# Autodesk Inventor assembly: assembly
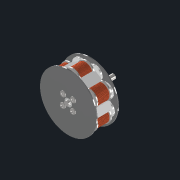
[picture p0: Inventor's stored thumbnail of the model, 180x180]
Saved by Autodesk Inventor 2022.2 (Build 262287010, 287A)
## iProperties
Created: 2023-07-19
Part Number: assembly
Document SubType Name: Assembly
Designer: StijnC
Author: StijnC
## Documents named in this file (10)
- C:\Users\techn\Desktop\AFM\V2\assembly.iam
- C:\Users\techn\Desktop\AFM\V2\motor15.ipt
- C:\Users\techn\Desktop\AFM\V2\core.ipt
- C:\Users\techn\Desktop\AFM\V2\magnet.ipt
- C:\Users\techn\Desktop\AFM\V2\plate.ipt
- C:\Users\techn\Desktop\AFM\V2\shaft.ipt
- C:\Users\techn\Desktop\AFM\V2\shaftmount.ipt
- C:\Users\techn\Desktop\AFM\V2\coil.ipt
- C:\Users\techn\Documents\Inventor\Content Center Files\R2022\en-US\DIN 625 - T1\DIN 625 T1 - 626 - 6 x 19 x 6.ipt
- C:\Users\techn\Documents\Inventor\Content Center Files\R2022\en-US\ANSI B18.3.4M(1)\ANSI B18.3.4M - M3 x 0.5 x 3(2).ipt
## Components (51 placed, 9 different names)
1. motor15:1 — Mate:1, Mate:2, Mate:3, Mate:6, Mate:7, Flush:1, Mate:30, Flush:2
2. motor15:2 — Mate:2, Mate:3, Mate:4, Mate:5, Angle:1, Flush:1, Mate:29, Flush:3
3. plate:1 — Mate:14, Mate:33, Mate:36, Mate:40, Insert:1, Insert:2, Insert:3, Insert:4
4. shaft:1 — Mate:14, Mate:15, Mate:31, Mate:32, Mate:41, Mate:43, Flush:4
5. plate:2 — Mate:15, Mate:18, Mate:19, Mate:34, Mate:37, Insert:5, Insert:6, Insert:7, Insert:8
6. shaftmount:1 — Mate:32, Mate:34, Mate:35, Mate:37, Mate:38, Angle:9
7. shaftmount:2 — Mate:31, Mate:33, Mate:35, Mate:36, Mate:39, Flush:4, Angle:7
8. DIN 625 - T1 626 - 6 x 19 x 6:1 — Mate:29, Flush:3, Mate:39
9. DIN 625 - T1 626 - 6 x 19 x 6:2 — Mate:30, Flush:2, Mate:38, Mate:43
10. Broached Hexagon Socket Button Head Cap Screw - Metric M3 x 0.5 x 3:1 — Insert:3, Angle:5, Angle:6
11. Broached Hexagon Socket Button Head Cap Screw - Metric M3 x 0.5 x 3:2 — Insert:1, Angle:6, Angle:7
12. Broached Hexagon Socket Button Head Cap Screw - Metric M3 x 0.5 x 3:3 — Insert:2, Angle:4
13. Broached Hexagon Socket Button Head Cap Screw - Metric M3 x 0.5 x 3:4 — Insert:4, Angle:4, Angle:5
14. Broached Hexagon Socket Button Head Cap Screw - Metric M3 x 0.5 x 3:5 — Insert:6, Angle:2, Angle:3
15. Broached Hexagon Socket Button Head Cap Screw - Metric M3 x 0.5 x 3:6 — Insert:5, Angle:2
16. Broached Hexagon Socket Button Head Cap Screw - Metric M3 x 0.5 x 3:7 — Insert:7, Angle:3, Angle:8, Angle:9
17. Broached Hexagon Socket Button Head Cap Screw - Metric M3 x 0.5 x 3:8 — Insert:8, Angle:8
18. core:2 — Mate:6, Mate:7
19. core:1 — Mate:4, Mate:5, Mate:28, Tangent:1
20. core:3
21. core:4
22. core:5
23. core:6
24. core:7
25. core:8
26. core:9
27. core:10
28. core:11
29. core:12
30. coil:1 — Mate:28, Tangent:1
31. coil:2
32. coil:3
33. coil:4
34. coil:5
35. coil:6
36. magnet:2 — Mate:18, Mate:19
37. magnet:3
38. magnet:4
39. magnet:5
40. magnet:6
41. magnet:7
42. magnet:8 — Mate:42
43. magnet:9
44. magnet:10 — Mate:40, Mate:41, Mate:42
45. magnet:11
46. magnet:12
47. magnet:13
48. magnet:14
49. magnet:15
50. magnet:16
51. magnet:17
## Component patterns: (6 elements, first: core:2 + core:1), (6 elements, first: coil:1), (8 elements, first: magnet:2), (8 elements, first: magnet:10)
## Relationships (49: Mate 27, Angle 9, Insert 8, Flush 4, Tangent 1)
- Mate:1: motor15:1
- Mate:2: motor15:1 ↔ motor15:2
- Mate:3: motor15:1 ↔ motor15:2
- Mate:4: motor15:2 ↔ core:1
- Mate:5: motor15:2 ↔ core:1
- Mate:6: motor15:1 ↔ core:2
- Mate:7: motor15:1 ↔ core:2
- Angle:1 (0 deg): motor15:2
- Flush:1: motor15:1 ↔ motor15:2
- Mate:14: plate:1 ↔ shaft:1
- Mate:15: shaft:1 ↔ plate:2
- Mate:18: plate:2 ↔ magnet:2
- Mate:19 (20.5 mm): plate:2 ↔ magnet:2
- Mate:28: core:1 ↔ coil:1
- Tangent:1: core:1 ↔ coil:1
- Mate:29: motor15:2 ↔ DIN 625 - T1 626 - 6 x 19 x 6:1
- Mate:30: motor15:1 ↔ DIN 625 - T1 626 - 6 x 19 x 6:2
- Flush:2: motor15:1 ↔ DIN 625 - T1 626 - 6 x 19 x 6:2
- Flush:3: motor15:2 ↔ DIN 625 - T1 626 - 6 x 19 x 6:1
- Mate:31: shaft:1 ↔ shaftmount:2
- Mate:32: shaft:1 ↔ shaftmount:1
- Mate:33: plate:1 ↔ shaftmount:2
- Mate:34: plate:2 ↔ shaftmount:1
- Mate:35: shaftmount:1 ↔ shaftmount:2
- Mate:36: plate:1 ↔ shaftmount:2
- Mate:37: plate:2 ↔ shaftmount:1
- Mate:38: shaftmount:1 ↔ DIN 625 - T1 626 - 6 x 19 x 6:2
- Mate:39: shaftmount:2 ↔ DIN 625 - T1 626 - 6 x 19 x 6:1
- Mate:40: plate:1 ↔ magnet:10
- Mate:41 (20.5 mm): shaft:1 ↔ magnet:10
- Mate:42: magnet:8 ↔ magnet:10
- Mate:43: shaft:1 ↔ DIN 625 - T1 626 - 6 x 19 x 6:2
- Flush:4 (-2 mm): shaft:1 ↔ shaftmount:2
- Insert:1: plate:1 ↔ Broached Hexagon Socket Button Head Cap Screw - Metric M3 x 0.5 x 3:2
- Insert:2: plate:1 ↔ Broached Hexagon Socket Button Head Cap Screw - Metric M3 x 0.5 x 3:3
- Insert:3: plate:1 ↔ Broached Hexagon Socket Button Head Cap Screw - Metric M3 x 0.5 x 3:1
- Insert:4: plate:1 ↔ Broached Hexagon Socket Button Head Cap Screw - Metric M3 x 0.5 x 3:4
- Insert:5: plate:2 ↔ Broached Hexagon Socket Button Head Cap Screw - Metric M3 x 0.5 x 3:6
- Insert:6: plate:2 ↔ Broached Hexagon Socket Button Head Cap Screw - Metric M3 x 0.5 x 3:5
- Insert:7: plate:2 ↔ Broached Hexagon Socket Button Head Cap Screw - Metric M3 x 0.5 x 3:7
- Insert:8: plate:2 ↔ Broached Hexagon Socket Button Head Cap Screw - Metric M3 x 0.5 x 3:8
- Angle:2 (0 deg): Broached Hexagon Socket Button Head Cap Screw - Metric M3 x 0.5 x 3:5 ↔ Broached Hexagon Socket Button Head Cap Screw - Metric M3 x 0.5 x 3:6
- Angle:3 (0 deg): Broached Hexagon Socket Button Head Cap Screw - Metric M3 x 0.5 x 3:5 ↔ Broached Hexagon Socket Button Head Cap Screw - Metric M3 x 0.5 x 3:7
- Angle:4 (0 deg): Broached Hexagon Socket Button Head Cap Screw - Metric M3 x 0.5 x 3:3 ↔ Broached Hexagon Socket Button Head Cap Screw - Metric M3 x 0.5 x 3:4
- Angle:5 (0 deg): Broached Hexagon Socket Button Head Cap Screw - Metric M3 x 0.5 x 3:1 ↔ Broached Hexagon Socket Button Head Cap Screw - Metric M3 x 0.5 x 3:4
- Angle:6 (0 deg): Broached Hexagon Socket Button Head Cap Screw - Metric M3 x 0.5 x 3:1 ↔ Broached Hexagon Socket Button Head Cap Screw - Metric M3 x 0.5 x 3:2
- Angle:7 (0 deg): shaftmount:2 ↔ Broached Hexagon Socket Button Head Cap Screw - Metric M3 x 0.5 x 3:2
- Angle:8 (0 deg): Broached Hexagon Socket Button Head Cap Screw - Metric M3 x 0.5 x 3:7 ↔ Broached Hexagon Socket Button Head Cap Screw - Metric M3 x 0.5 x 3:8
- Angle:9 (0 deg): shaftmount:1 ↔ Broached Hexagon Socket Button Head Cap Screw - Metric M3 x 0.5 x 3:7
